# Autodesk Inventor assembly: Assembly3
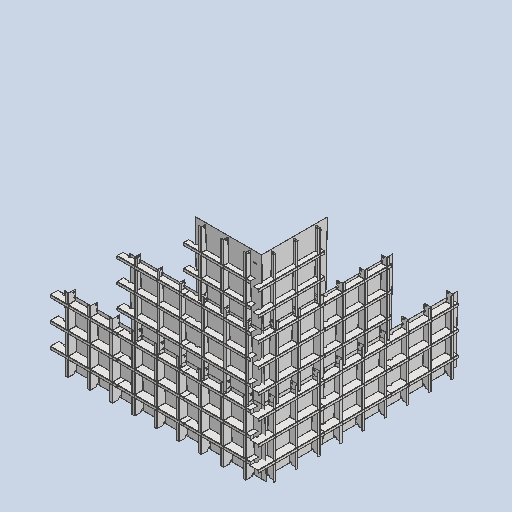
[picture p0: Inventor's stored thumbnail of the model, 512x512]
Saved by Autodesk Inventor 2026 (Build 300175000, 175)
## iProperties
Created: 2026-06-02
Part Number: Assembly3
Document SubType Name: Assembly
Designer: admin
Author: admin
## Documents named in this file (9)
- C:\Users\pokla\Documents\Inventor\GBK-Gubkinskiy\Assembly3.iam
- C:\Users\pokla\Documents\Inventor\GBK-Gubkinskiy\ASY GBK 2130 short wall shield 3.iam
- C:\Users\pokla\Documents\Inventor\GBK-Gubkinskiy\ASY GBK 2330 short wall shield 9.iam
- C:\Users\pokla\Documents\Inventor\GBK-Gubkinskiy\ASY GBK 2120 short wall shield 2.iam
- C:\Users\pokla\Documents\Inventor\GBK-Gubkinskiy\ASY GBK 2230 short wall shield 6.iam
- C:\Users\pokla\Documents\Inventor\GBK-Gubkinskiy\ASY GBK 1110 long wall shield 1.iam
- C:\Users\pokla\Documents\Inventor\GBK-Gubkinskiy\ASY GBK 1210 long wall shield 3.iam
- C:\Users\pokla\Documents\Inventor\GBK-Gubkinskiy\ASY GBK 1310 long wall shield 4.iam
- C:\Users\pokla\Documents\Inventor\GBK-Gubkinskiy\ASY GBK 1120 long wall shield 2.iam
## Components (8 placed, 8 different names)
1. ASY GBK 2130 short wall shield 3:1 [sub-assembly] — Заподлицо:3, Совмещение:2, Заподлицо:4, Совмещение:3
2. ASY GBK 2330 short wall shield 7:1 [sub-assembly] — Заподлицо:5, Совмещение:4, Совмещение:5
3. ASY GBK 2120 short wall shield 2:1 [sub-assembly]
4. ASY GBK 2230 short wall shield 6:1 [sub-assembly] — Заподлицо:4, Совмещение:3, Заподлицо:5, Совмещение:4, Совмещение:5
5. ASY GBK 1110 long wall shield 1:1 [sub-assembly] — Заподлицо:1, Совмещение:1, Заподлицо:2
6. 04 ASY GBK wall shield 1.2.4:1 [sub-assembly]
7. 07 ASY GBK wall shield 1.3.1:1 [sub-assembly]
8. 02 ASY GBK wall shield 1.1.2:1 [sub-assembly]
## Relationships (14: Flush 5, Mate 5, WeldJoint 4)
- [WeldJoint] (1 mm): ASY GBK 2130 short wall shield 3:1 ↔ ASY GBK 2120 short wall shield 2:1
- [WeldJoint]: ASY GBK 1110 long wall shield 1:1 ↔ 04 ASY GBK wall shield 1.2.4:1
- [WeldJoint]: 04 ASY GBK wall shield 1.2.4:1 ↔ 07 ASY GBK wall shield 1.3.1:1
- [WeldJoint] (1 mm): ASY GBK 1110 long wall shield 1:1 ↔ 02 ASY GBK wall shield 1.1.2:1
- Заподлицо:1 [Flush]: ASY GBK 1110 long wall shield 1:1
- Совмещение:1 [Mate]: ASY GBK 1110 long wall shield 1:1
- Заподлицо:2 [Flush]: ASY GBK 1110 long wall shield 1:1
- Заподлицо:3 [Flush]: ASY GBK 2130 short wall shield 3:1
- Совмещение:2 [Mate] (100 mm): ASY GBK 2130 short wall shield 3:1
- Заподлицо:4 [Flush]: ASY GBK 2130 short wall shield 3:1 ↔ ASY GBK 2230 short wall shield 6:1
- Совмещение:3 [Mate] (1 mm): ASY GBK 2130 short wall shield 3:1 ↔ ASY GBK 2230 short wall shield 6:1
- Заподлицо:5 [Flush]: ASY GBK 2330 short wall shield 7:1 ↔ ASY GBK 2230 short wall shield 6:1
- Совмещение:4 [Mate] (1 mm): ASY GBK 2330 short wall shield 7:1 ↔ ASY GBK 2230 short wall shield 6:1
- Совмещение:5 [Mate] (1 mm): ASY GBK 2330 short wall shield 7:1 ↔ ASY GBK 2230 short wall shield 6:1
